# Autodesk Inventor assembly: Assembly3
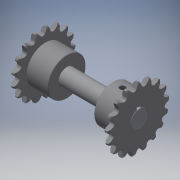
[picture p0: Inventor's stored thumbnail of the model, 180x180]
Saved by Autodesk Inventor 2019 (Build 230136000, 136)
## iProperties
Created: 2021-08-30
Part Number: Assembly3
Material: 一般
Document SubType Name: Assembly
Designer: yuta
Author: yuta
## Documents named in this file (3)
- C:\Users\yuta\Documents\キャチロボ\Assembly3.iam
- C:\Users\yuta\Documents\AIS2019\SUSFBN25B17D10_().ipt
- C:\Users\yuta\Documents\キャチロボ\Part16.ipt
## Components (3 placed, 2 different names)
1. SUSFBN25B17D10_():1 — メイト:1, メイト:2
2. SUSFBN25B17D10_():2 — メイト:3, メイト:4
3. Part16:1 — メイト:1, メイト:2, メイト:3, メイト:4
## Relationships (4: Mate 4)
- メイト:1 [Mate]: SUSFBN25B17D10_():1 ↔ Part16:1
- メイト:2 [Mate]: SUSFBN25B17D10_():1 ↔ Part16:1
- メイト:3 [Mate]: SUSFBN25B17D10_():2 ↔ Part16:1
- メイト:4 [Mate]: SUSFBN25B17D10_():2 ↔ Part16:1
